# Autodesk Inventor assembly: kciuk
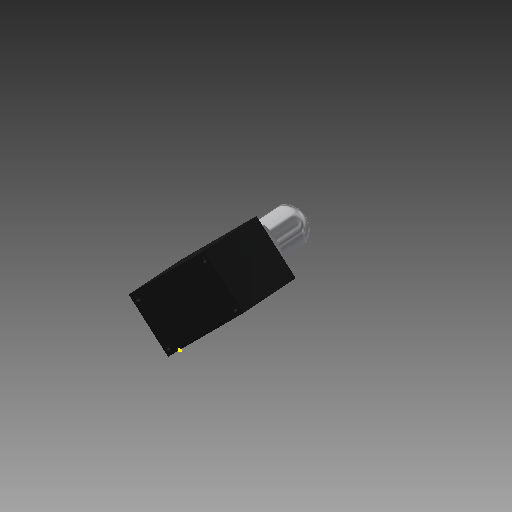
[picture p0: Inventor's stored thumbnail of the model, 512x512]
Saved by Autodesk Inventor 2019 (Build 230136000, 136)
## iProperties
Created: 2019-11-26
Part Number: kciuk
Document SubType Name: Assembly
Designer: Administrator
Title: *New thumb whole v3
Author: Administrator
## Documents named in this file (9)
- C:\Users\Karolina\Desktop\Kuba\rekav2\kciuk\kciuk.iam
- C:\Users\Karolina\Desktop\Kuba\rekav2\fiusion360\Hand show version v5 v4.f3d v1\Middle (1) (1).ipt
- C:\Users\Karolina\Desktop\Kuba\rekav2\fiusion360\Hand show version v5 v4.f3d v1\Tip (1) (1).ipt
- C:\Users\Karolina\Desktop\Kuba\rekav2\fiusion360\Hand show version v5 v4.f3d v1\Lever (4).ipt
- C:\Users\Karolina\Desktop\Kuba\rekav2\fiusion360\Hand show version v5 v4.f3d v1\Body (9).ipt
- C:\Users\Karolina\Desktop\Kuba\rekav2\fiusion360\Hand show version v5 v4.f3d v1\Base (4).ipt
- C:\Users\Karolina\Desktop\Kuba\rekav2\kciuk\Pulley_small.ipt
- C:\Users\Karolina\Desktop\Kuba\rekav2\kciuk\Pullie.ipt
- C:\Users\Karolina\Desktop\Kuba\rekav2\kciuk\Servo.ipt
## Components (10 placed, 8 different names)
1. Middle (1) (1):1 — Zestawiający:3, Zestawiający:4, Zestawiający:7, Zestawiający:9
2. Tip (1) (1):1 — Zestawiający:7, Zestawiający:8, Zestawiający:9
3. Lever (4):1 — Zestawiający:5, Zestawiający:6, Zestawiający:8
4. Body (9):1 — Zestawiający:1, Zestawiający:2, Zestawiający:10, Zestawiający:11, Zestawiający:12, Zestawiający:13, Zestawiający:14, Zestawiający:15, Zestawiający:16, Zestawiający:17, Zestawiający:18, Zestawiający:19, Zestawiający:20
5. Base (4):1 — Zestawiający:1, Zestawiający:2, Zestawiający:3, Zestawiający:4, Zestawiający:5, Zestawiający:6
6. Pulley_small:1 — Zestawiający:13, Zestawiający:15
7. Pullie:1 — Zestawiający:10, Zestawiający:17
8. Pulley_small:2 — Zestawiający:12, Zestawiający:14
9. Pullie:2 — Zestawiający:11, Zestawiający:16
10. Servo:1 — Zestawiający:18, Zestawiający:19, Zestawiający:20
## Relationships (20: Mate 20)
- Zestawiający:1 [Mate]: Body (9):1 ↔ Base (4):1
- Zestawiający:2 [Mate]: Body (9):1 ↔ Base (4):1
- Zestawiający:3 [Mate]: Middle (1) (1):1 ↔ Base (4):1
- Zestawiający:4 [Mate]: Middle (1) (1):1 ↔ Base (4):1
- Zestawiający:5 [Mate]: Lever (4):1 ↔ Base (4):1
- Zestawiający:6 [Mate]: Lever (4):1 ↔ Base (4):1
- Zestawiający:7 [Mate]: Middle (1) (1):1 ↔ Tip (1) (1):1
- Zestawiający:8 [Mate]: Tip (1) (1):1 ↔ Lever (4):1
- Zestawiający:9 [Mate]: Middle (1) (1):1 ↔ Tip (1) (1):1
- Zestawiający:10 [Mate]: Body (9):1 ↔ Pullie:1
- Zestawiający:11 [Mate]: Body (9):1 ↔ Pullie:2
- Zestawiający:12 [Mate]: Body (9):1 ↔ Pulley_small:2
- Zestawiający:13 [Mate]: Body (9):1 ↔ Pulley_small:1
- Zestawiający:14 [Mate]: Body (9):1 ↔ Pulley_small:2
- Zestawiający:15 [Mate]: Body (9):1 ↔ Pulley_small:1
- Zestawiający:16 [Mate]: Body (9):1 ↔ Pullie:2
- Zestawiający:17 [Mate]: Body (9):1 ↔ Pullie:1
- Zestawiający:18 [Mate]: Body (9):1 ↔ Servo:1
- Zestawiający:19 [Mate]: Body (9):1 ↔ Servo:1
- Zestawiający:20 [Mate]: Body (9):1 ↔ Servo:1
